# Autodesk Inventor assembly: ScannerMountingOption1
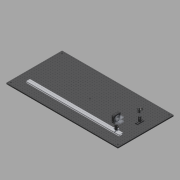
[picture p0: Inventor's stored thumbnail of the model, 180x180]
Saved by Autodesk Inventor 2018 (Build 220112000, 112)
## iProperties
Created: 2018-09-17
Part Number: ScannerMountingOption1
Document SubType Name: Assembly
Designer: Robert Campbell
Author: Robert Campbell
## Documents named in this file (5)
- X:\home\work\Documents\MF_BenchOptics\CAD_files\ScannerMountingOption1.iam
- X:\home\work\Documents\MF_BenchOptics\CAD_files\MB60120_M-Solidworks.ipt
- X:\home\work\Documents\MF_BenchOptics\CAD_files\XT66DP-1000-Solidworks.ipt
- X:\home\work\Documents\MF_BenchOptics\CAD_files\first_mirror.iam
- W:\home\work\Documents\MF_BenchOptics\CAD_files\MountedScanners.iam
## Components (4 placed, 4 different names)
1. MB60120_M-Solidworks:1 — Mate:1, Mate:21
2. XT66DP-1000-Solidworks:1 — Mate:1, Angle:1, Mate:22
3. first_mirror:1 [sub-assembly] — Mate:21
4. MountedScanners:1 [sub-assembly] — Angle:1, Mate:22
## Relationships (4: Mate 3, Angle 1)
- Mate:1: MB60120_M-Solidworks:1 ↔ XT66DP-1000-Solidworks:1
- Mate:21: MB60120_M-Solidworks:1 ↔ first_mirror:1
- Angle:1 (0 deg): XT66DP-1000-Solidworks:1 ↔ MountedScanners:1
- Mate:22: XT66DP-1000-Solidworks:1 ↔ MountedScanners:1
